# Autodesk Inventor assembly: WholeModelCarbonFiber
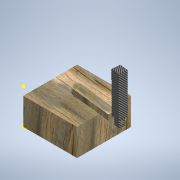
[picture p0: Inventor's stored thumbnail of the model, 180x180]
Saved by Autodesk Inventor 2021 (Build 250183000, 183)
## iProperties
Created: 2022-10-04
Part Number: WholeModelCarbonFiber
Document SubType Name: Assembly
Designer: mrizw
Author: mrizw
## Documents named in this file (4)
- D:\ElectroMechanicalSystems\AutoCad\WholeModelCarbonFiber.iam
- D:\ElectroMechanicalSystems\AutoCad\Base.ipt
- D:\ElectroMechanicalSystems\AutoCad\Arm.ipt
- D:\ElectroMechanicalSystems\AutoCad\Pendulum.ipt
## Components (3 placed, 3 different names)
1. Base:1 — Rotational:1
2. Arm:1 — Rotational:1, Rotational:2
3. Pendulum:1 — Rotational:2
## Relationships (2: RevoluteJoint 2)
- Rotational:1 [RevoluteJoint]: Base:1 ↔ Arm:1
- Rotational:2 [RevoluteJoint]: Arm:1 ↔ Pendulum:1
